# Autodesk Inventor assembly: Assembly1
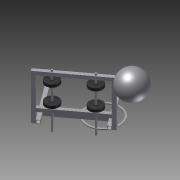
[picture p0: Inventor's stored thumbnail of the model, 180x180]
Saved by Autodesk Inventor 2011 SP1 (Build 150282100, 282)
## iProperties
Created: 2012-01-14
Part Number: Assembly1
Document SubType Name: Assembly
Designer: Christopher
Author: Christopher
## Documents named in this file (9)
- C:\Users\Christopher\Documents\Christopher\FIRST\Inventor files\2012\4 wheel kicker version 1\Assembly1.iam
- C:\Users\Christopher\Documents\Christopher\FIRST\Inventor files\2012\4 wheel kicker version 1\9 in .125 aluminum tube.ipt
- C:\Users\Christopher\Documents\Christopher\FIRST\Inventor files\2012\4 wheel kicker version 1\18 inch tube.ipt
- C:\Users\Christopher\Documents\Christopher\FIRST\Inventor files\2012\4 wheel kicker version 1\wheel.ipt
- C:\Users\Christopher\Documents\Christopher\FIRST\Inventor files\2012\4 wheel kicker version 1\axle1 .5inch.ipt
- C:\Users\Christopher\Documents\Christopher\FIRST\Inventor files\2012\4 wheel kicker version 1\game ball.ipt
- C:\Users\Christopher\Documents\Christopher\FIRST\Inventor files\2012\4 wheel kicker version 1\16.25inch tube.ipt
- C:\Users\Christopher\Documents\Christopher\FIRST\Inventor files\2012\4 wheel kicker version 1\proxyturntable.ipt
- C:\Users\Christopher\Documents\Christopher\FIRST\Inventor files\2012\4 wheel kicker version 1\14.25inch tube.ipt
## Components (15 placed, 8 different names)
1. 18 inch tube:2 — Insert:1, Insert:2, Mate:1, Flush:1, Flush:2, Flush:3, Mate:6
2. wheel:1 — Insert:3
3. wheel:2 — Insert:4
4. wheel:3 — Insert:9
5. wheel:4 — Insert:10
6. axle1 .5inch:1 — Insert:1, Insert:3, Insert:9, Insert:11
7. axle1 .5inch:2 — Insert:2, Insert:4, Insert:10
8. game ball:1
9. 9 in .125 aluminum tube:1 — Mate:1, Flush:1, Flush:2, Mate:4, Insert:12
10. 16.25inch tube:1 — Insert:11, Mate:4, Mate:5, Tangent:1
11. proxyturntable:1 — Mate:8, Tangent:1
12. 9 in .125 aluminum tube:2 — Mate:5, Flush:3, Mate:6, Insert:13
13. 9 in .125 aluminum tube:3 — Insert:12, Flush:6
14. 9 in .125 aluminum tube:4 — Insert:13, Mate:7, Flush:4, Flush:5
15. 14.25inch tube:1 — Mate:7, Flush:4, Flush:5, Flush:6, Mate:8
## Relationships (22: Insert 9, Mate 6, Flush 6, Tangent 1)
- Insert:1 (-12.7 mm): 18 inch tube:2 ↔ axle1 .5inch:1
- Insert:2 (-12.7 mm): 18 inch tube:2 ↔ axle1 .5inch:2
- Insert:3 (66.04 mm): wheel:1 ↔ axle1 .5inch:1
- Insert:4 (66.04 mm): wheel:2 ↔ axle1 .5inch:2
- Mate:1: 18 inch tube:2 ↔ 9 in .125 aluminum tube:1
- Flush:1: 18 inch tube:2 ↔ 9 in .125 aluminum tube:1
- Flush:2: 18 inch tube:2 ↔ 9 in .125 aluminum tube:1
- Insert:9 (205.74 mm): wheel:3 ↔ axle1 .5inch:1
- Insert:10 (205.74 mm): wheel:4 ↔ axle1 .5inch:2
- Insert:11 (254 mm): axle1 .5inch:1 ↔ 16.25inch tube:1
- Mate:4: 9 in .125 aluminum tube:1 ↔ 16.25inch tube:1
- Mate:5: 16.25inch tube:1 ↔ 9 in .125 aluminum tube:2
- Flush:3: 18 inch tube:2 ↔ 9 in .125 aluminum tube:2
- Mate:6: 18 inch tube:2 ↔ 9 in .125 aluminum tube:2
- Insert:12: 9 in .125 aluminum tube:1 ↔ 9 in .125 aluminum tube:3
- Insert:13: 9 in .125 aluminum tube:2 ↔ 9 in .125 aluminum tube:4
- Mate:7: 9 in .125 aluminum tube:4 ↔ 14.25inch tube:1
- Flush:4: 9 in .125 aluminum tube:4 ↔ 14.25inch tube:1
- Flush:5 (76.2 mm): 9 in .125 aluminum tube:4 ↔ 14.25inch tube:1
- Flush:6: 9 in .125 aluminum tube:3 ↔ 14.25inch tube:1
- Mate:8: proxyturntable:1 ↔ 14.25inch tube:1
- Tangent:1: 16.25inch tube:1 ↔ proxyturntable:1
